# Autodesk Inventor assembly: Foot_MIR
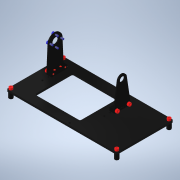
[picture p0: Inventor's stored thumbnail of the model, 180x180]
Saved by Autodesk Inventor 2022 (Build 260153000, 153)
## iProperties
Created: 2022-06-04
Part Number: Foot_MIR
Document SubType Name: Assembly
Designer: Masato Kubotera
Author: Masato Kubotera
## Documents named in this file (9)
- C:\Users\MasatoKubotera\Desktop\SUSTAINA-OP\LowerBody\Foot\Foot_MIR.iam
- C:\Users\MasatoKubotera\Desktop\SUSTAINA-OP\LowerBody\Foot\Sole_frame.ipt
- C:\Users\MasatoKubotera\Desktop\SUSTAINA-OP\LowerBody\Foot\Foot_front_frame.ipt
- C:\Users\MasatoKubotera\Desktop\SUSTAINA-OP\LowerBody\Foot\Foot_back_frame.ipt
- C:\Users\MasatoKubotera\Desktop\SUSTAINA-OP\LowerBody\Foot\Foot_root_block.ipt
- C:\Users\MasatoKubotera\Desktop\SUSTAINA-OP\ReadyMade\Spacer\ASL-309BE.ipt
- C:\Users\MasatoKubotera\Desktop\SUSTAINA-OP\ReadyMade\Screw\UC-0310.ipt
- C:\Users\MasatoKubotera\Desktop\SUSTAINA-OP\ReadyMade\Screw\UC-0308.ipt
- C:\Users\MasatoKubotera\Desktop\SUSTAINA-OP\ReadyMade\Screw\UC-2606.ipt
## Components (25 placed, 8 different names)
1. Sole_frame:1 — 挿入:2, 挿入:1, 挿入:4, 挿入:3, 挿入:13, 挿入:14, 挿入:15, 挿入:16, 挿入:21, 挿入:22, 挿入:23, 挿入:24, 挿入:25, 挿入:26, 挿入:27, 挿入:28
2. Foot_front_frame:1 — メイト:2, メイト:1, 挿入:6, 挿入:5, 挿入:31, 挿入:32
3. Foot_back_frame:1 — 挿入:8, 挿入:7, 挿入:29, 挿入:30, 挿入:33, 挿入:34, 挿入:35, 挿入:36
4. Foot_root_block:1 — 挿入:6, 挿入:5, 挿入:2, 挿入:1
5. Foot_root_block:2 — 挿入:8, 挿入:7, 挿入:4, 挿入:3
6. UC-2606:1 — 挿入:33
7. UC-2606:2 — 挿入:34
8. UC-2606:3 — 挿入:35
9. UC-2606:4 — 挿入:36
10. ASL-309BE:1 — メイト:3, 挿入:21, 角度:1
11. ASL-309BE:2 — 挿入:22, 角度:2
12. ASL-309BE:3 — 挿入:23, 角度:3
13. ASL-309BE:4 — 挿入:24, 角度:4
14. UC-0310:1 — 挿入:25
15. UC-0310:2 — 挿入:26
16. UC-0310:3 — 挿入:27
17. UC-0310:4 — 挿入:28
18. UC-0308:1 — 挿入:13
19. UC-0308:2 — 挿入:14
20. UC-0308:3 — 挿入:15
21. UC-0308:4 — 挿入:16
22. UC-0308:5 — 挿入:32
23. UC-0308:6 — 挿入:31
24. UC-0308:7 — 挿入:30
25. UC-0308:8 — 挿入:29
## Relationships (35: Insert 28, Angle 4, Mate 3)
- メイト:2 [Mate]: Foot_front_frame:1
- メイト:1 [Mate]: Foot_front_frame:1
- 挿入:6 [Insert]: Foot_front_frame:1 ↔ Foot_root_block:1
- 挿入:5 [Insert]: Foot_front_frame:1 ↔ Foot_root_block:1
- 挿入:2 [Insert]: Sole_frame:1 ↔ Foot_root_block:1
- 挿入:1 [Insert]: Sole_frame:1 ↔ Foot_root_block:1
- 挿入:8 [Insert]: Foot_back_frame:1 ↔ Foot_root_block:2
- 挿入:7 [Insert]: Foot_back_frame:1 ↔ Foot_root_block:2
- 挿入:4 [Insert]: Sole_frame:1 ↔ Foot_root_block:2
- 挿入:3 [Insert]: Sole_frame:1 ↔ Foot_root_block:2
- 挿入:13 [Insert]: Sole_frame:1 ↔ UC-0308:1
- 挿入:14 [Insert]: Sole_frame:1 ↔ UC-0308:2
- 挿入:15 [Insert]: Sole_frame:1 ↔ UC-0308:3
- 挿入:16 [Insert]: Sole_frame:1 ↔ UC-0308:4
- メイト:3 [Mate]: ASL-309BE:1
- 挿入:21 [Insert]: Sole_frame:1 ↔ ASL-309BE:1
- 挿入:22 [Insert]: Sole_frame:1 ↔ ASL-309BE:2
- 挿入:23 [Insert]: Sole_frame:1 ↔ ASL-309BE:3
- 挿入:24 [Insert]: Sole_frame:1 ↔ ASL-309BE:4
- 挿入:25 [Insert]: Sole_frame:1 ↔ UC-0310:1
- 挿入:26 [Insert]: Sole_frame:1 ↔ UC-0310:2
- 挿入:27 [Insert]: Sole_frame:1 ↔ UC-0310:3
- 挿入:28 [Insert]: Sole_frame:1 ↔ UC-0310:4
- 挿入:29 [Insert]: Foot_back_frame:1 ↔ UC-0308:8
- 挿入:30 [Insert]: Foot_back_frame:1 ↔ UC-0308:7
- 挿入:31 [Insert]: Foot_front_frame:1 ↔ UC-0308:6
- 挿入:32 [Insert]: Foot_front_frame:1 ↔ UC-0308:5
- 角度:1 [Angle] (0 deg): ASL-309BE:1
- 角度:2 [Angle] (0 deg): ASL-309BE:2
- 角度:3 [Angle] (0 deg): ASL-309BE:3
- 角度:4 [Angle] (0 deg): ASL-309BE:4
- 挿入:33 [Insert]: Foot_back_frame:1 ↔ UC-2606:1
- 挿入:34 [Insert]: Foot_back_frame:1 ↔ UC-2606:2
- 挿入:35 [Insert]: Foot_back_frame:1 ↔ UC-2606:3
- 挿入:36 [Insert]: Foot_back_frame:1 ↔ UC-2606:4
